# Autodesk Inventor assembly: PEEK Cutout
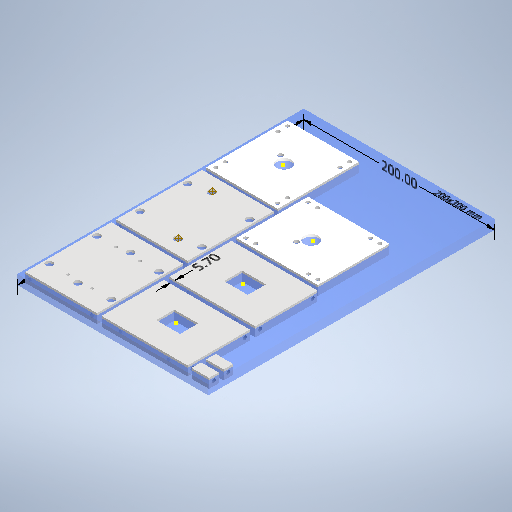
[picture p0: Inventor's stored thumbnail of the model, 512x512]
Saved by Autodesk Inventor 2025.3 (Build 293356000, 356)
## iProperties
Created: 2025-05-16
Part Number: PEEK Cutout
Document SubType Name: Assembly
Designer: Verðandi
Author: Verðandi
## Documents named in this file (7)
- E:\Users\USER\Documents\GitHub\LAFriOC\Rb oven\Rb PEEK\PEEK Cutout.iam
- E:\Users\USER\Documents\GitHub\LAFriOC\Rb oven\Rb PEEK\Rb PEEK - Arriba.ipt
- E:\Users\USER\Documents\GitHub\LAFriOC\Rb oven\Rb PEEK\Rb PEEK - Corto.ipt
- E:\Users\USER\Documents\GitHub\LAFriOC\Rb oven\Rb PEEK\Rb PEEK - Largo.ipt
- E:\Users\USER\Documents\GitHub\LAFriOC\Rb oven\Rb PEEK\Rb PEEK - Soporte.ipt
- E:\Users\USER\Documents\GitHub\LAFriOC\Rb oven\Rb PEEK\Rb PEEK - Abajo_MIR.ipt
- E:\Users\USER\Documents\GitHub\LAFriOC\Rb oven\Rb PEEK\PEEK Sheet.ipt
## Components (9 placed, 6 different names)
1. PEEK Sheet:1
2. Rb PEEK - Arriba:1 — Mate:1, Mate:2
3. Rb PEEK - Corto:1 — Mate:5
4. Rb PEEK - Largo:1 — Mate:3, Mate:4, Mate:6
5. Rb PEEK - Soporte:1 — Mate:7
6. Rb PEEK - Abajo_MIR:1 — Mate:2, Mate:3
7. Rb PEEK - Corto:2 — Mate:1
8. Rb PEEK - Largo:2 — Mate:4, Mate:5
9. Rb PEEK - Soporte:2 — Mate:6, Mate:7
## Relationships (7: Mate 7)
- Mate:1: Rb PEEK - Arriba:1 ↔ Rb PEEK - Corto:2
- Mate:2: Rb PEEK - Arriba:1 ↔ Rb PEEK - Abajo_MIR:1
- Mate:3: Rb PEEK - Largo:1 ↔ Rb PEEK - Abajo_MIR:1
- Mate:4: Rb PEEK - Largo:1 ↔ Rb PEEK - Largo:2
- Mate:5: Rb PEEK - Corto:1 ↔ Rb PEEK - Largo:2
- Mate:6: Rb PEEK - Largo:1 ↔ Rb PEEK - Soporte:2
- Mate:7: Rb PEEK - Soporte:1 ↔ Rb PEEK - Soporte:2
